# Autodesk Inventor assembly: Zespół1
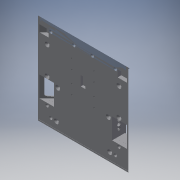
[picture p0: Inventor's stored thumbnail of the model, 180x180]
Saved by Autodesk Inventor 2019 (Build 230136000, 136)
## iProperties
Created: 2021-11-14
Part Number: Zespół1
Material: Ogólny
Document SubType Name: Assembly
Designer: Michał
Author: Michał
## Documents named in this file (15)
- D:\Projekty\RoboIlo\ninja\Zespół1.iam
- D:\Projekty\RoboIlo\ninja\blacha.ipt
- D:\Projekty\RoboIlo\ninja\mocowanie_silnika_wariant1.ipt
- D:\Projekty\RoboIlo\ninja\MocowanieCzujnikaBezScianki.ipt
- D:\Projekty\RoboIlo\ninja\MocowanieBok2.ipt
- D:\Projekty\RoboIlo\ninja\mocowanie_silnika_wariant1_MIR.ipt
- D:\Projekty\RoboIlo\ninja\MocowanieBok2_MIR.ipt
- D:\Projekty\RoboIlo\ninja\MocowanieCzujnikaBazSciankiLewy.ipt
- D:\Projekty\RoboIlo\ninja\Bok2mm.ipt
- D:\Projekty\RoboIlo\ninja\Przod2mm.ipt
- D:\Projekty\RoboIlo\ninja\Bok2mm_MIR.ipt
- D:\Projekty\RoboIlo\ninja\Tyl2.ipt
- D:\Projekty\RoboIlo\ninja\PLUG.ipt
- D:\Projekty\RoboIlo\ninja\PlogPiramida.ipt
- D:\Projekty\RoboIlo\ninja\Dach2.ipt
## Components (14 placed, 14 different names)
1. blacha:1 — Wstaw:1, Wstaw:2, Wstaw:6, Zestawiający:1, Zestawiający:2, Zestawiający:3, Wstaw:19, Wstaw:20, Wstaw:27, Wstaw:28, Wstaw:29, Wstaw:30, Wstaw:39, Wstaw:40, Wstaw:41, Wstaw:42
2. MocowanieCzujnikaBezScianki:1 — Wstaw:1, Wstaw:2, Wstaw:5, Wstaw:37, Wstaw:38
3. mocowanie_silnika_wariant1:1 — Wstaw:5, Wstaw:6, Wstaw:35
4. MocowanieBok2:1 — Wstaw:27, Wstaw:28
5. mocowanie_silnika_wariant1_MIR:1 — Wstaw:19, Wstaw:21, Wstaw:36, Równoległy:1
6. MocowanieBok2_MIR:1 — Wstaw:29, Wstaw:30
7. MocowanieCzujnikaBazSciankiLewy:1 — Wstaw:20, Wstaw:21, Wstaw:31, Wstaw:32, Wstaw:33, Wstaw:34
8. Bok2mm:1 — Wstaw:33, Wstaw:34
9. Przod2mm:1 — Wstaw:31, Wstaw:32
10. Bok2mm_MIR:1 — Wstaw:37, Wstaw:38
11. Tyl2:1 — Wstaw:35, Wstaw:36
12. PLUG:1 — Wstaw:39, Wstaw:40
13. PlogPiramida:1 — Wstaw:41, Wstaw:42
14. Dach2:1 — Równoległy:1
## Relationships (27: Insert 23, Mate 3, Flush 1)
- Wstaw:1 [Insert]: blacha:1 ↔ MocowanieCzujnikaBezScianki:1
- Wstaw:2 [Insert]: blacha:1 ↔ MocowanieCzujnikaBezScianki:1
- Wstaw:5 [Insert]: MocowanieCzujnikaBezScianki:1 ↔ mocowanie_silnika_wariant1:1
- Wstaw:6 [Insert]: blacha:1 ↔ mocowanie_silnika_wariant1:1
- Zestawiający:1 [Mate]: blacha:1
- Zestawiający:2 [Mate]: blacha:1
- Zestawiający:3 [Mate]: blacha:1
- Wstaw:19 [Insert]: blacha:1 ↔ mocowanie_silnika_wariant1_MIR:1
- Wstaw:20 [Insert]: blacha:1 ↔ MocowanieCzujnikaBazSciankiLewy:1
- Wstaw:21 [Insert]: mocowanie_silnika_wariant1_MIR:1 ↔ MocowanieCzujnikaBazSciankiLewy:1
- Wstaw:27 [Insert]: blacha:1 ↔ MocowanieBok2:1
- Wstaw:28 [Insert]: blacha:1 ↔ MocowanieBok2:1
- Wstaw:29 [Insert]: blacha:1 ↔ MocowanieBok2_MIR:1
- Wstaw:30 [Insert]: blacha:1 ↔ MocowanieBok2_MIR:1
- Wstaw:31 [Insert]: MocowanieCzujnikaBazSciankiLewy:1 ↔ Przod2mm:1
- Wstaw:32 [Insert]: MocowanieCzujnikaBazSciankiLewy:1 ↔ Przod2mm:1
- Wstaw:33 [Insert]: MocowanieCzujnikaBazSciankiLewy:1 ↔ Bok2mm:1
- Wstaw:34 [Insert]: MocowanieCzujnikaBazSciankiLewy:1 ↔ Bok2mm:1
- Wstaw:35 [Insert]: mocowanie_silnika_wariant1:1 ↔ Tyl2:1
- Wstaw:36 [Insert]: mocowanie_silnika_wariant1_MIR:1 ↔ Tyl2:1
- Wstaw:37 [Insert]: MocowanieCzujnikaBezScianki:1 ↔ Bok2mm_MIR:1
- Wstaw:38 [Insert]: MocowanieCzujnikaBezScianki:1 ↔ Bok2mm_MIR:1
- Wstaw:39 [Insert]: blacha:1 ↔ PLUG:1
- Wstaw:40 [Insert]: blacha:1 ↔ PLUG:1
- Wstaw:41 [Insert]: blacha:1 ↔ PlogPiramida:1
- Wstaw:42 [Insert]: blacha:1 ↔ PlogPiramida:1
- Równoległy:1 [Flush]: mocowanie_silnika_wariant1_MIR:1 ↔ Dach2:1
